# Autodesk Inventor assembly: A1-18002-150-00 Line boring skid weldment
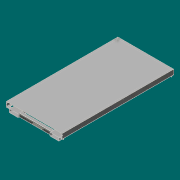
[picture p0: Inventor's stored thumbnail of the model, 180x180]
Saved by Autodesk Inventor 2017 (Build 210142000, 142)
## iProperties
Created: 2018-01-23
Part Number: A1-18002-150-00 Line boring skid weldment
Document SubType Name: Weldment
Designer: Graeme_Van_Dongen
Mass: 2.94826e+06 g
Surface Area: 313203 cm^2
Volume: 587682 cm^3
Density: 5.01675 g/cm^3
Weld Material: Steel, Mild, Welded
_SolveAssemblyDoc: Frame Generator Solve Assembly
_Version: 15.0.0
Author: Graeme_Van_Dongen
## Documents named in this file (6)
- N:\A1 - Projects\A1-18\A1-18002--Alco Line boring skid\A1-18002-150-00 Line boring skid weldment.iam
- N:\A1 - Projects\A1-18\A1-18002--Alco Line boring skid\A1-18002-100-01 Floor.ipt
- N:\A1 - Projects\A1-18\A1-18002--Alco Line boring skid\Base frame skeleton.ipt
- N:\A1 - Projects\A1-18\A1-18002--Alco Line boring skid\A1-18002-100-00 Line boring skid\Frame\Frame0001.iam
- N:\A1 - Projects\A1-18\A1-18002--Alco Line boring skid\A1-18002-100-38 Leg hinge pin.ipt
- N:\Inventor\Content Center Files\R2017\en-US\ANSI AISC(2)\AISC - 2 1_2x1_4 - 2.ipt
## Components (11 placed, 5 different names)
1. A1-18002-100-01 Floor:1 — Flush:7, Flush:8, Flush:9, Flush:30, Flush:31, Flush:32
2. Base frame skeleton:1 — Flush:30, Flush:31, Flush:32
3. Frame0001:1 [sub-assembly] — Insert:58, Angle:37, Insert:59, Mate:22, Mate:23, Flush:36, Mate:24, Flush:37, Flush:38
4. A1-18002-100-38 Leg hinge pin:1 — Insert:58, Angle:37, Angle:38
5. A1-18002-100-38 Leg hinge pin:2 — Insert:59, Angle:38
6. ANSI AISC (Rectangular) 2 1/2x1/4 - 2:1 — Mate:22, Mate:23, Flush:36
7. ANSI AISC (Rectangular) 2 1/2x1/4 - 2:2 — Mate:24, Flush:37, Flush:38
8. A1-18002-100-38 Leg hinge pin:3
9. A1-18002-100-38 Leg hinge pin:4
10. ANSI AISC (Rectangular) 2 1/2x1/4 - 2:3
11. ANSI AISC (Rectangular) 2 1/2x1/4 - 2:4
## Component patterns: (2 elements, first: A1-18002-100-38 Leg hinge pin:1 + A1-18002-100-38 Leg hinge pin:2 + ANSI AISC (Rectangular) 2 1/2x1/4 - 2:1 + ANSI AISC (Rectangular) 2 1/2x1/4 - 2:2)
## Relationships (16: Flush 9, Mate 3, Insert 2, Angle 2)
- Flush:7: A1-18002-100-01 Floor:1
- Flush:8: A1-18002-100-01 Floor:1
- Flush:9: A1-18002-100-01 Floor:1
- Flush:30: A1-18002-100-01 Floor:1 ↔ Base frame skeleton:1
- Flush:31: A1-18002-100-01 Floor:1 ↔ Base frame skeleton:1
- Flush:32 (101.6 mm): A1-18002-100-01 Floor:1 ↔ Base frame skeleton:1
- Insert:58: Frame0001:1 ↔ A1-18002-100-38 Leg hinge pin:1
- Angle:37 (0 deg): Frame0001:1 ↔ A1-18002-100-38 Leg hinge pin:1
- Insert:59: Frame0001:1 ↔ A1-18002-100-38 Leg hinge pin:2
- Angle:38 (0 deg): A1-18002-100-38 Leg hinge pin:1 ↔ A1-18002-100-38 Leg hinge pin:2
- Mate:22: Frame0001:1 ↔ ANSI AISC (Rectangular) 2 1/2x1/4 - 2:1
- Mate:23: Frame0001:1 ↔ ANSI AISC (Rectangular) 2 1/2x1/4 - 2:1
- Flush:36: Frame0001:1 ↔ ANSI AISC (Rectangular) 2 1/2x1/4 - 2:1
- Mate:24: Frame0001:1 ↔ ANSI AISC (Rectangular) 2 1/2x1/4 - 2:2
- Flush:37: Frame0001:1 ↔ ANSI AISC (Rectangular) 2 1/2x1/4 - 2:2
- Flush:38: Frame0001:1 ↔ ANSI AISC (Rectangular) 2 1/2x1/4 - 2:2
